# Autodesk Inventor assembly: MotorBlock
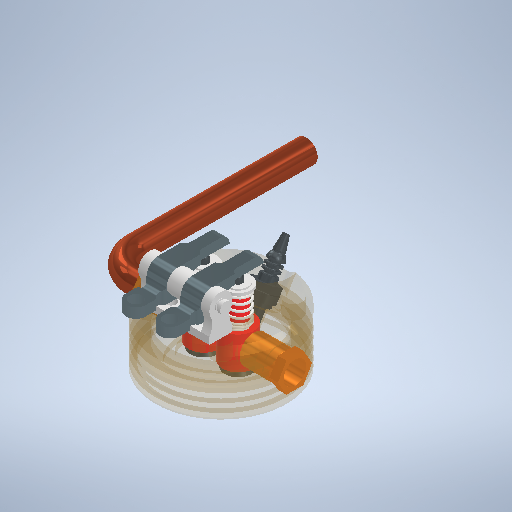
[picture p0: Inventor's stored thumbnail of the model, 512x512]
Saved by Autodesk Inventor 2025 (Build 290162010, 162A)
## iProperties
Created: 2024-07-16
Part Number: MotorBlock
Document SubType Name: Assembly
Designer: ffogue
Author: ffogue
## Documents named in this file (13)
- C:\Users\ffogue\OneDrive - MuM - OM\Dokumente\Inventor\Boxermotor\MotorBlock.iam
- C:\Users\ffogue\OneDrive - MuM - OM\Dokumente\Inventor\Boxermotor\Ventil.ipt
- C:\Users\ffogue\OneDrive - MuM - OM\Dokumente\Inventor\Boxermotor\KopmressionsFeder_ventil.ipt
- C:\Users\ffogue\OneDrive - MuM - OM\Dokumente\Inventor\Boxermotor\ventiltasse.ipt
- C:\Users\ffogue\OneDrive - MuM - OM\Dokumente\Inventor\Boxermotor\deckeGehaeuse.ipt
- C:\Users\ffogue\OneDrive - MuM - OM\Dokumente\Inventor\Boxermotor\kipphebellagerbock.ipt
- C:\Users\ffogue\OneDrive - MuM - OM\Dokumente\Inventor\Boxermotor\Kipphebelachse.ipt
- C:\Users\ffogue\OneDrive - MuM - OM\Dokumente\Inventor\Boxermotor\KippHebel.ipt
- C:\Users\ffogue\OneDrive - MuM - OM\Dokumente\Inventor\Boxermotor\distanzbüchse_kipphebel.ipt
- C:\Users\ffogue\OneDrive - MuM - OM\Dokumente\Inventor\Boxermotor\überwurfmutter.ipt
- C:\Users\ffogue\OneDrive - MuM - OM\Dokumente\Inventor\Boxermotor\Auspuffkrümmer.ipt
- C:\Users\ffogue\OneDrive - MuM - OM\Dokumente\Inventor\Boxermotor\zündkerze.ipt
- C:\Users\ffogue\OneDrive - MuM - OM\Dokumente\Inventor\Boxermotor\Miederhalter_ventilfeder.ipt
## Components (18 placed, 12 different names)
1. Ventil:2 — Mate:6, Insert:18, Insert:37
2. Compress Spring1:2 — Mate:8, Cylindrical:2
3. ventiltasse:1 — Mate:4, Insert:17, Mate:6, Insert:18, Mate:8, Cylindrical:2
4. ventiltasse:2 — Mate:3, Insert:16, Mate:7, Insert:19, Mate:9, Cylindrical:3, Angle:3, Mate:19, Insert:29
5. deckeGehaeuse:1 — Mate:3, Mate:4, Insert:16, Insert:17, Mate:10, Mate:11, Insert:22, Angle:1, Angle:2, Mate:16, Mate:17, Insert:27, Insert:28, Mate:18, Mate:21, Insert:30
6. Ventil:3 — Mate:7, Insert:19, Insert:36
7. Compress Spring1:3 — Mate:9, Cylindrical:3
8. kipphebellagerbock:1 — Mate:10, Mate:11, Insert:22, Mate:12, Insert:23, Insert:24
9. Kipphebelachse:1 — Mate:12, Insert:23, Mate:13, Mate:14, Mate:15
10. KippHebel:1 — Mate:13, Insert:24, Insert:25, Angle:1
11. KippHebel:2 — Mate:15, Insert:26, Angle:2
12. distanzbüchse_kipphebel:1 — Mate:14, Insert:25, Insert:26
13. überwurfmutter:2 — Mate:16, Insert:28
14. überwurfmutter:3 — Mate:17, Insert:27
15. Auspuffkrümmer:1 — Mate:20, Insert:29
16. zündkerze:1 — Mate:21, Insert:30
17. Miederhalter_ventilfeder:1 — Insert:36
18. Miederhalter_ventilfeder:2 — Insert:37
## Relationships (38: Mate 18, Insert 15, Angle 3, CylindricalJoint 2)
- Mate:3: ventiltasse:2 ↔ deckeGehaeuse:1
- Mate:4: ventiltasse:1 ↔ deckeGehaeuse:1
- Insert:16: ventiltasse:2 ↔ deckeGehaeuse:1
- Insert:17: ventiltasse:1 ↔ deckeGehaeuse:1
- Mate:6: Ventil:2 ↔ ventiltasse:1
- Insert:18 (-2 mm): Ventil:2 ↔ ventiltasse:1
- Mate:7: ventiltasse:2 ↔ Ventil:3
- Insert:19 (-2 mm): ventiltasse:2 ↔ Ventil:3
- Mate:8: Compress Spring1:2 ↔ ventiltasse:1
- Mate:9: ventiltasse:2 ↔ Compress Spring1:3
- Cylindrical:2: Compress Spring1:2 ↔ ventiltasse:1
- Cylindrical:3: ventiltasse:2 ↔ Compress Spring1:3
- Mate:10: deckeGehaeuse:1 ↔ kipphebellagerbock:1
- Mate:11: deckeGehaeuse:1 ↔ kipphebellagerbock:1
- Insert:22: deckeGehaeuse:1 ↔ kipphebellagerbock:1
- Mate:12: kipphebellagerbock:1 ↔ Kipphebelachse:1
- Insert:23 (-26.5 mm): kipphebellagerbock:1 ↔ Kipphebelachse:1
- Mate:13: Kipphebelachse:1 ↔ KippHebel:1
- Insert:24: kipphebellagerbock:1 ↔ KippHebel:1
- Mate:14: Kipphebelachse:1 ↔ distanzbüchse_kipphebel:1
- Insert:25: KippHebel:1 ↔ distanzbüchse_kipphebel:1
- Mate:15: Kipphebelachse:1 ↔ KippHebel:2
- Insert:26: KippHebel:2 ↔ distanzbüchse_kipphebel:1
- Angle:1 (180 deg): deckeGehaeuse:1 ↔ KippHebel:1
- Angle:2 (180 deg): deckeGehaeuse:1 ↔ KippHebel:2
- Mate:16: deckeGehaeuse:1 ↔ überwurfmutter:2
- Mate:17: deckeGehaeuse:1 ↔ überwurfmutter:3
- Insert:27 (3 mm): deckeGehaeuse:1 ↔ überwurfmutter:3
- Insert:28 (3 mm): deckeGehaeuse:1 ↔ überwurfmutter:2
- Mate:18: deckeGehaeuse:1
- Angle:3 (90 deg): ventiltasse:2
- Mate:19: ventiltasse:2
- Mate:20: Auspuffkrümmer:1
- Insert:29: ventiltasse:2 ↔ Auspuffkrümmer:1
- Mate:21: deckeGehaeuse:1 ↔ zündkerze:1
- Insert:30: deckeGehaeuse:1 ↔ zündkerze:1
- Insert:36: Ventil:3 ↔ Miederhalter_ventilfeder:1
- Insert:37: Ventil:2 ↔ Miederhalter_ventilfeder:2
